# Autodesk Inventor assembly: RBPB5
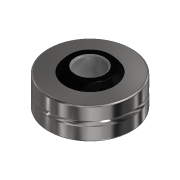
[picture p0: Inventor's stored thumbnail of the model, 180x180]
Saved by Autodesk Inventor 2021 (Build 250183000, 183)
## iProperties
Part Number: RBPB5
Catalog Web Link: www.cadenas.de
Description: RBPB-Spherical Bearings - Standard Type
Vendor: MISUMI
Document SubType Name: Assembly
Designer: partserver
Manufacturer: MISUMI
Mass: 1.1592 g
Surface Area: 12.2353 cm^2
Volume: 1.1592 cm^3
Density: 1 g/cm^3
Category: PARTsolutions
Company: MISUMI
PSOL_IDENT_0: {$CADENAS_DATA\23d-libs\misumi\metric\34_cylinders\rbpb_asmtab.prj},153 {VTYP=3D},{STYP=ASSTAB},{NB=
PSOL_IDENT_1: RBPB5},{LINA=RBPB5},{NN=RBPB},{DATE=30.06.2021 13:14:18},{GEOMDATE=11.07.2011},{VERSION=},{LINEID=10
PSOL_IDENT_2: },{WBVAR=},{WBNUMERIC=}  {NB=RBPB5},{LINA=RBPB5},{KT=DUMMY},{PN=RBPB5},{TYPE=RBPB},{MATH=1035 Steel}
PSOL_IDENT_3: ,{MATSIR=51200 Bearing Steel},{STSIR=Hard Chrome Plating},{HARDSIR=58HRC~},{MATB=Special Copper Allo
PSOL_IDENT_4: y},{DD=5},{D=16},{B=6.00},{B1=8},{DD1=7.7},{H=1.0},{R=0.3},{BD=11.112},{A1=8},{A11=8},{A2=13},{A3=30
PSOL_IDENT_5: },{SLC=7.84},{SLC1=7.84},{MASS=8.5},{RDC=0.035mm or Less},{ADC=0.1mm or Less},{PPATH=rbpb_asmtpl.prj
PSOL_IDENT_6: }
NB: RBPB5
NN: RBPB
NT: Spherical Bearings - Standard Type
NBSYN: $PN.
LINA: RBPB5
CATALOG: Misumi
PN: RBPB5
MATH: 1035 Steel
MATSIR: 51200 Bearing Steel
STSIR: Hard Chrome Plating
HARDSIR: 58HRC~
MATB: Special Copper Alloy
DD: 5
D: 16
B: 6
B1: 8
DD1: 7.7
H: 1
R: 0.3
BD: 11.112
A1: 8
A2: 13
A3: 30
SLC: 7.84
MASS: 8.5
RDC: 0.035mm or Less
ADC: 0.1mm or Less
SUPPLIER: MISUMI
ARTICLENO: RBPB5
BOMINFO: RBPB5
CREATOR: CADENAS GmbH
Title: RBPB5
Author: Cadenas PARTsolutions
Comments: Spherical Bearings - Standard Type
## Documents named in this file (4)
- C:\Users\Rama\Desktop\Voron-2-2.4r1\Custom\Misumi GE5C\RBPB5-Bearing\RBPB5.iam
- C:\Users\Rama\Desktop\Voron-2-2.4r1\Custom\Misumi GE5C\RBPB5-Bearing\RBPB5dummy.ipt
- C:\Users\Rama\Desktop\Voron-2-2.4r1\Custom\Misumi GE5C\RBPB5-Bearing\RBPB5h.ipt
- C:\Users\Rama\Desktop\Voron-2-2.4r1\Custom\Misumi GE5C\RBPB5-Bearing\RBPB5ball.ipt
## Components (3 placed, 3 different names)
1. RBPB5dummy:1 — dummy_Z@1 <-> holder_Z@2
2. RBPB5h:1 — dummy_Z@1 <-> holder_Z@2, holder_Z@2 <-> ball_Z@3
3. RBPB5ball:1 — holder_Z@2 <-> ball_Z@3
## Relationships (2: Mate 2)
- dummy_Z@1 <-> holder_Z@2 [Mate]: RBPB5dummy:1 ↔ RBPB5h:1
- holder_Z@2 <-> ball_Z@3 [Mate]: RBPB5h:1 ↔ RBPB5ball:1
